# Autodesk Inventor assembly: CCM_Unit
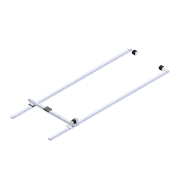
[picture p0: Inventor's stored thumbnail of the model, 180x180]
Saved by Autodesk Inventor 2020 (Build 240168000, 168)
## iProperties
Created: 2021-02-24
Part Number: CCM_Unit
Document SubType Name: Assembly
Designer: magnarecta
Author: magnarecta
## Documents named in this file (8)
- D:\Document\Github\Eto_Project\Hardware\Asem\CCM_Unit.iam
- D:\Document\Github\Eto_Project\Hardware\Parts\CCM\CCM motion linear guide rail\CCM_UNIT\CCM_Unit_C.iam
- D:\Document\Github\Eto_Project\Hardware\Parts\CCM\CCM motion linear guide rail\CCM_UNIT\CCM_Unit_A.iam
- D:\Document\Github\Eto_Project\Hardware\Parts\CCM\CCM motion linear guide rail\CCM_UNIT\CCM_Unit_B.iam
- D:\Document\Github\Eto_Project\Hardware\Parts\Meviy\CCM_Mount_A.ipt
- D:\Document\Github\Eto_Project\Hardware\Parts\CCM\CCM motion linear guide rail\57 Aside Speed Reducer(2050)__1.ipt
- D:\Document\Github\Eto_Project\Hardware\Parts\Stepper_Motor\NEMA23 Stepper.ipt
- D:\Document\Github\Eto_Project\Hardware\Parts\Meviy\CCM_Mount_B.ipt
## Components (9 placed, 7 different names)
1. CCM_Unit_C:1 [sub-assembly] — メイト:1, 角度:1, メイト:3, フラッシュ:8, 挿入:5, 挿入:6, フラッシュ:10, フラッシュ:11
2. CCM_Unit_A:1 [sub-assembly] — フラッシュ:1, フラッシュ:2, フラッシュ:3, フラッシュ:4, メイト:1, 角度:1, 挿入:3, 挿入:4, 挿入:8
3. CCM_Unit_B:1 [sub-assembly] — フラッシュ:1, フラッシュ:2, フラッシュ:3, フラッシュ:4, 挿入:9, 角度:3, 挿入:10, 挿入:11
4. CCM_Mount_A:2 — メイト:3, 挿入:3, 挿入:4, フラッシュ:8
5. 57 Aside Speed Reducer(2050)__1:1 — 挿入:5, 挿入:6, 挿入:7, 角度:2
6. NEMA23 Stepper:1 — 挿入:7, 角度:2
7. NEMA23 Stepper:2 — 挿入:9, 角度:3, フラッシュ:9
8. NEMA23 Stepper:3 — 挿入:8, フラッシュ:9
9. CCM_Mount_B:1 — 挿入:10, 挿入:11, フラッシュ:10, フラッシュ:11
## Relationships (22: Insert 9, Flush 8, Angle 3, Mate 2)
- フラッシュ:1 [Flush]: CCM_Unit_A:1 ↔ CCM_Unit_B:1
- フラッシュ:2 [Flush]: CCM_Unit_A:1 ↔ CCM_Unit_B:1
- フラッシュ:3 [Flush]: CCM_Unit_A:1 ↔ CCM_Unit_B:1
- フラッシュ:4 [Flush]: CCM_Unit_A:1 ↔ CCM_Unit_B:1
- メイト:1 [Mate] (3 mm): CCM_Unit_C:1 ↔ CCM_Unit_A:1
- 角度:1 [Angle] (0 deg): CCM_Unit_C:1 ↔ CCM_Unit_A:1
- メイト:3 [Mate]: CCM_Unit_C:1 ↔ CCM_Mount_A:2
- 挿入:3 [Insert]: CCM_Unit_A:1 ↔ CCM_Mount_A:2
- 挿入:4 [Insert]: CCM_Unit_A:1 ↔ CCM_Mount_A:2
- フラッシュ:8 [Flush]: CCM_Unit_C:1 ↔ CCM_Mount_A:2
- 挿入:5 [Insert]: CCM_Unit_C:1 ↔ 57 Aside Speed Reducer(2050)__1:1
- 挿入:6 [Insert]: CCM_Unit_C:1 ↔ 57 Aside Speed Reducer(2050)__1:1
- 挿入:7 [Insert]: 57 Aside Speed Reducer(2050)__1:1 ↔ NEMA23 Stepper:1
- 角度:2 [Angle] (0 deg): 57 Aside Speed Reducer(2050)__1:1 ↔ NEMA23 Stepper:1
- 挿入:8 [Insert] (2 mm): CCM_Unit_A:1 ↔ NEMA23 Stepper:3
- 挿入:9 [Insert] (2 mm): CCM_Unit_B:1 ↔ NEMA23 Stepper:2
- 角度:3 [Angle] (0 deg): CCM_Unit_B:1 ↔ NEMA23 Stepper:2
- フラッシュ:9 [Flush]: NEMA23 Stepper:2 ↔ NEMA23 Stepper:3
- 挿入:10 [Insert]: CCM_Unit_B:1 ↔ CCM_Mount_B:1
- 挿入:11 [Insert]: CCM_Unit_B:1 ↔ CCM_Mount_B:1
- フラッシュ:10 [Flush] (20 mm): CCM_Unit_C:1 ↔ CCM_Mount_B:1
- フラッシュ:11 [Flush]: CCM_Unit_C:1 ↔ CCM_Mount_B:1
